# Autodesk Inventor assembly: Heatbed Sandwich
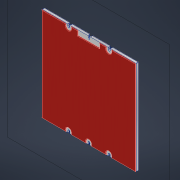
[picture p0: Inventor's stored thumbnail of the model, 180x180]
Saved by Autodesk Inventor 2022.2 (Build 262287010, 287A)
## iProperties
Created: 2022-03-13
Part Number: Heatbed Sandwich
Document SubType Name: Assembly
Designer: sleib
Author: sleib
## Documents named in this file (4)
- C:\Users\sleib\Projekte\Voron-2\CAD\Inventor\Heatbed Sandwich.iam
- C:\Users\sleib\Projekte\Voron-2\CAD\Inventor\Heatbed.ipt
- C:\Users\sleib\Projekte\Voron-2\CAD\Inventor\Heatbed Magnetic-Sheet.ipt
- C:\Users\sleib\Projekte\Voron-2\CAD\Inventor\Silicon-Heater (350mm).ipt
## Components (3 placed, 3 different names)
1. Heatbed:1 — Fluchtend:1, Passend:1, Passend:2, Fluchtend:2
2. Heatbed Magnetic-Sheet:1 — Fluchtend:1
3. Silicon-Heater (350mm):1 — Passend:1, Passend:2, Fluchtend:2
## Relationships (4: Flush 2, Mate 2)
- Fluchtend:1 [Flush]: Heatbed:1 ↔ Heatbed Magnetic-Sheet:1
- Passend:1 [Mate]: Heatbed:1 ↔ Silicon-Heater (350mm):1
- Passend:2 [Mate]: Heatbed:1 ↔ Silicon-Heater (350mm):1
- Fluchtend:2 [Flush]: Heatbed:1 ↔ Silicon-Heater (350mm):1
